# Autodesk Inventor assembly: Laufkatze_Baugruppe_neu
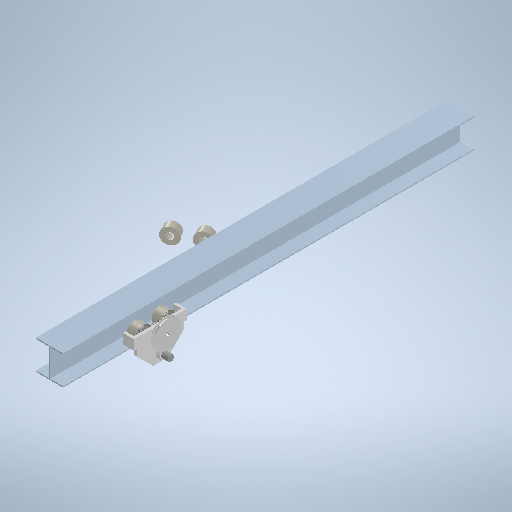
[picture p0: Inventor's stored thumbnail of the model, 512x512]
Saved by Autodesk Inventor 2025.2 (Build 292293000, 293)
## iProperties
Created: 2025-02-05
Part Number: Laufkatze_Baugruppe_neu
Document SubType Name: Assembly
Designer: akoca
Author: akoca
## Documents named in this file (11)
- C:\Users\akoca\Documents\MCI\Semester_3\AMEII\Projekt\Laufkatze\Baugruppen\Laufkatze_Baugruppe_neu.iam
- C:\Users\akoca\Documents\MCI\Semester_3\AMEII\Projekt\Laufkatze\Einzelbauteile\Stahlträger.ipt
- C:\Users\akoca\Documents\MCI\Semester_3\AMEII\Projekt\Laufkatze\Einzelbauteile\Zahnrad_für_Kettenzug.ipt
- C:\Users\akoca\Documents\MCI\Semester_3\AMEII\Projekt\Laufkatze\Einzelbauteile\Zahnrad_bei_Laufrad.ipt
- C:\Users\akoca\Documents\MCI\Semester_3\AMEII\Projekt\Laufkatze\Einzelbauteile\Laufrad.ipt
- C:\Users\akoca\Documents\MCI\Semester_3\AMEII\Projekt\Laufkatze\Einzelbauteile\Welle_für_Kettenzug.ipt
- C:\Users\akoca\Documents\MCI\Semester_3\AMEII\Projekt\Laufkatze\Einzelbauteile\Führungsplatte_rechts.ipt
- C:\Users\akoca\Documents\MCI\Semester_3\AMEII\Projekt\Laufkatze\Baugruppen\Laufkatze_Baugruppe\Konstruktions-Assistent\Lager4.iam
- C:\Users\akoca\Documents\MCI\Semester_3\AMEII\Projekt\Laufkatze\Einzelbauteile\Zugscheibe_für_Kette.ipt
- C:\Users\akoca\Documents\MCI\Semester_3\AMEII\Projekt\Laufkatze\Einzelbauteile\Führungsplatte_links.ipt
- C:\Users\akoca\Documents\MCI\Semester_3\AMEII\Projekt\Laufkatze\Einzelbauteile\Schraubbolzen.ipt
## Components (15 placed, 10 different names)
1. Stahlträger:1 — Tangential:3, Tangential:4, Passend:5, Passend:6, Drehung/Translation:1, Tangential:5, Tangential:6, Passend:9
2. Zahnrad_für_Kettenzug:1 — Fluchtend:1, Fluchtend:2, Tangential:1, Tangential:2, Drehung:1, Drehung:2, Zahnrad-Bewegung, Drehung:3
3. Zahnrad_bei_Laufrad:1 — Fluchtend:1, Tangential:2, Passend:2, Starr:2, Drehbar:7, Drehung:1
4. Zahnrad_bei_Laufrad:2 — Fluchtend:2, Tangential:1, Passend:4, Starr:1, Drehbar:8, Drehung:2
5. Laufrad:1 — Passend:4, Tangential:4, Starr:1, Passend:5, Drehung/Translation:1
6. Laufrad:2 — Passend:2, Tangential:3, Starr:2, Passend:6
7. Welle_für_Kettenzug:1 — Starr:4, Starr:5, Zahnrad-Bewegung, Drehbar:9
8. Führungsplatte_rechts:1 — Drehbar:8, Drehbar:7, Passend:7
9. Lager:1 [sub-assembly] — Starr:4
10. Lager:2 [sub-assembly] — Starr:5
11. Zugscheibe_für_Kette:1 — Drehbar:9, Drehung:3
12. Führungsplatte_links:1 — Drehbar:12, Drehbar:13, Passend:8
13. Laufrad:3 — Drehbar:13, Tangential:5, Passend:9
14. Laufrad:4 — Drehbar:12, Tangential:6
15. Schraubbolzen:1 — Passend:7, Passend:8
## Relationships (29: Mate 7, Tangent 6, RevoluteJoint 6, WeldJoint 4, RelateRotation 3, Flush 2, RelateRotateTranslate 1)
- Fluchtend:1 [Flush]: Zahnrad_für_Kettenzug:1 ↔ Zahnrad_bei_Laufrad:1
- Fluchtend:2 [Flush]: Zahnrad_für_Kettenzug:1 ↔ Zahnrad_bei_Laufrad:2
- Tangential:1: Zahnrad_für_Kettenzug:1 ↔ Zahnrad_bei_Laufrad:2
- Tangential:2: Zahnrad_für_Kettenzug:1 ↔ Zahnrad_bei_Laufrad:1
- Passend:2 [Mate]: Zahnrad_bei_Laufrad:1 ↔ Laufrad:2
- Passend:4 [Mate]: Zahnrad_bei_Laufrad:2 ↔ Laufrad:1
- Tangential:3: Stahlträger:1 ↔ Laufrad:2
- Tangential:4: Stahlträger:1 ↔ Laufrad:1
- Starr:1 [WeldJoint]: Zahnrad_bei_Laufrad:2 ↔ Laufrad:1
- Starr:2 [WeldJoint]: Zahnrad_bei_Laufrad:1 ↔ Laufrad:2
- Drehbar:8 [RevoluteJoint] (2 mm): Zahnrad_bei_Laufrad:2 ↔ Führungsplatte_rechts:1
- Drehbar:7 [RevoluteJoint] (2 mm): Zahnrad_bei_Laufrad:1 ↔ Führungsplatte_rechts:1
- Passend:5 [Mate]: Stahlträger:1 ↔ Laufrad:1
- Passend:6 [Mate]: Stahlträger:1 ↔ Laufrad:2
- Drehung:1 [RelateRotation] (0.6 ul): Zahnrad_für_Kettenzug:1 ↔ Zahnrad_bei_Laufrad:1
- Drehung:2 [RelateRotation] (0.6 ul): Zahnrad_für_Kettenzug:1 ↔ Zahnrad_bei_Laufrad:2
- Starr:4 [WeldJoint]: Welle_für_Kettenzug:1 ↔ Lager:1
- Starr:5 [WeldJoint]: Welle_für_Kettenzug:1 ↔ Lager:2
- Zahnrad-Bewegung [RevoluteJoint]: Zahnrad_für_Kettenzug:1 ↔ Welle_für_Kettenzug:1
- Drehbar:9 [RevoluteJoint]: Welle_für_Kettenzug:1 ↔ Zugscheibe_für_Kette:1
- Drehung:3 [RelateRotation] (1 ul): Zahnrad_für_Kettenzug:1 ↔ Zugscheibe_für_Kette:1
- Drehung/Translation:1 [RelateRotateTranslate] (339.292 mm): Stahlträger:1 ↔ Laufrad:1
- Drehbar:12 [RevoluteJoint] (2 mm): Führungsplatte_links:1 ↔ Laufrad:4
- Drehbar:13 [RevoluteJoint]: Führungsplatte_links:1 ↔ Laufrad:3
- Passend:7 [Mate]: Führungsplatte_rechts:1 ↔ Schraubbolzen:1
- Passend:8 [Mate]: Führungsplatte_links:1 ↔ Schraubbolzen:1
- Tangential:5: Stahlträger:1 ↔ Laufrad:3
- Tangential:6: Stahlträger:1 ↔ Laufrad:4
- Passend:9 [Mate]: Stahlträger:1 ↔ Laufrad:3
